# Autodesk Inventor assembly: Kühler_hinten
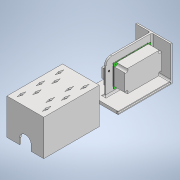
[picture p0: Inventor's stored thumbnail of the model, 180x180]
Saved by Autodesk Inventor 2021 (Build 250183000, 183)
## iProperties
Created: 2021-11-08
Part Number: Kühler_hinten
Document SubType Name: Assembly
Designer: Simon
Author: Simon
## Documents named in this file (8)
- C:\WORK\MILK_COOLER\milk_cooler\cad\Kühler_hinten.iam
- C:\WORK\MILK_COOLER\milk_cooler\cad\netzteil_12V.ipt
- C:\WORK\MILK_COOLER\milk_cooler\cad\netzteil_5V.ipt
- C:\WORK\MILK_COOLER\milk_cooler\cad\netzteil_halter_unten.ipt
- C:\WORK\MILK_COOLER\milk_cooler\cad\distanzhalter_schraube.ipt
- C:\Users\simub\Documents\Inventor\Content Center Files\R2021\de-DE\DIN EN ISO 4035\DIN EN ISO 4035 - M2.5.ipt
- C:\WORK\MILK_COOLER\milk_cooler\cad\relais.ipt
- C:\WORK\MILK_COOLER\milk_cooler\cad\netzteil_halter_oben.ipt
## Components (25 placed, 7 different names)
1. netzteil_12V:1 — Einfügen:6, Passend:1
2. netzteil_5V:1 — Einfügen:19, Passend:2
3. netzteil_halter_unten:1 — Fluchtend:1, Fluchtend:2, Fluchtend:3, Einfügen:2, Einfügen:3, Einfügen:4, Einfügen:5, Einfügen:7, Einfügen:8, Einfügen:9, Einfügen:10, Einfügen:11, Einfügen:12, Einfügen:13, Einfügen:14, Einfügen:15, Einfügen:16, Einfügen:17, Einfügen:18, Einfügen:22, Einfügen:23, Einfügen:25, Einfügen:26, Passend:4, Passend:5
4. distanzhalter_schraube:1 — Einfügen:5, Einfügen:6
5. distanzhalter_schraube:2 — Einfügen:2
6. distanzhalter_schraube:3 — Einfügen:4
7. distanzhalter_schraube:4 — Einfügen:3, Passend:1
8. distanzhalter_schraube:5 — Einfügen:11, Einfügen:19
9. DIN EN ISO 4035 M2.5:1 — Einfügen:9
10. DIN EN ISO 4035 M2.5:2 — Einfügen:10
11. DIN EN ISO 4035 M2.5:3 — Einfügen:8
12. DIN EN ISO 4035 M2.5:4 — Einfügen:7
13. distanzhalter_schraube:6 — Einfügen:14, Passend:2
14. distanzhalter_schraube:7 — Einfügen:13
15. distanzhalter_schraube:8 — Einfügen:12
16. DIN EN ISO 4035 M2.5:5 — Einfügen:16
17. DIN EN ISO 4035 M2.5:6 — Einfügen:18
18. DIN EN ISO 4035 M2.5:7 — Einfügen:17
19. DIN EN ISO 4035 M2.5:8 — Einfügen:15
20. relais:1 — Einfügen:24, Passend:3
21. distanzhalter_schraube:9 — Einfügen:23, Einfügen:24
22. distanzhalter_schraube:10 — Einfügen:22, Passend:3
23. DIN EN ISO 4035 M2.5:9 — Einfügen:25
24. DIN EN ISO 4035 M2.5:10 — Einfügen:26
25. netzteil_halter_oben:1 — Passend:4, Passend:5
## Relationships (31: Insert 23, Mate 5, Flush 3)
- Fluchtend:1 [Flush]: netzteil_halter_unten:1
- Fluchtend:2 [Flush]: netzteil_halter_unten:1
- Fluchtend:3 [Flush]: netzteil_halter_unten:1
- Einfügen:2 [Insert]: netzteil_halter_unten:1 ↔ distanzhalter_schraube:2
- Einfügen:3 [Insert]: netzteil_halter_unten:1 ↔ distanzhalter_schraube:4
- Einfügen:4 [Insert]: netzteil_halter_unten:1 ↔ distanzhalter_schraube:3
- Einfügen:5 [Insert]: netzteil_halter_unten:1 ↔ distanzhalter_schraube:1
- Einfügen:6 [Insert]: netzteil_12V:1 ↔ distanzhalter_schraube:1
- Passend:1 [Mate]: netzteil_12V:1 ↔ distanzhalter_schraube:4
- Einfügen:7 [Insert]: netzteil_halter_unten:1 ↔ DIN EN ISO 4035 M2.5:4
- Einfügen:8 [Insert]: netzteil_halter_unten:1 ↔ DIN EN ISO 4035 M2.5:3
- Einfügen:9 [Insert]: netzteil_halter_unten:1 ↔ DIN EN ISO 4035 M2.5:1
- Einfügen:10 [Insert]: netzteil_halter_unten:1 ↔ DIN EN ISO 4035 M2.5:2
- Einfügen:11 [Insert]: netzteil_halter_unten:1 ↔ distanzhalter_schraube:5
- Einfügen:12 [Insert]: netzteil_halter_unten:1 ↔ distanzhalter_schraube:8
- Einfügen:13 [Insert]: netzteil_halter_unten:1 ↔ distanzhalter_schraube:7
- Einfügen:14 [Insert]: netzteil_halter_unten:1 ↔ distanzhalter_schraube:6
- Einfügen:15 [Insert]: netzteil_halter_unten:1 ↔ DIN EN ISO 4035 M2.5:8
- Einfügen:16 [Insert]: netzteil_halter_unten:1 ↔ DIN EN ISO 4035 M2.5:5
- Einfügen:17 [Insert]: netzteil_halter_unten:1 ↔ DIN EN ISO 4035 M2.5:7
- Einfügen:18 [Insert]: netzteil_halter_unten:1 ↔ DIN EN ISO 4035 M2.5:6
- Einfügen:19 [Insert]: netzteil_5V:1 ↔ distanzhalter_schraube:5
- Passend:2 [Mate]: netzteil_5V:1 ↔ distanzhalter_schraube:6
- Einfügen:22 [Insert]: netzteil_halter_unten:1 ↔ distanzhalter_schraube:10
- Einfügen:23 [Insert]: netzteil_halter_unten:1 ↔ distanzhalter_schraube:9
- Einfügen:24 [Insert]: relais:1 ↔ distanzhalter_schraube:9
- Passend:3 [Mate]: relais:1 ↔ distanzhalter_schraube:10
- Einfügen:25 [Insert]: netzteil_halter_unten:1 ↔ DIN EN ISO 4035 M2.5:9
- Einfügen:26 [Insert]: netzteil_halter_unten:1 ↔ DIN EN ISO 4035 M2.5:10
- Passend:4 [Mate] (0.5 mm): netzteil_halter_unten:1 ↔ netzteil_halter_oben:1
- Passend:5 [Mate] (0.5 mm): netzteil_halter_unten:1 ↔ netzteil_halter_oben:1
